# Autodesk Inventor assembly: Custom Cover Full Assembly_2
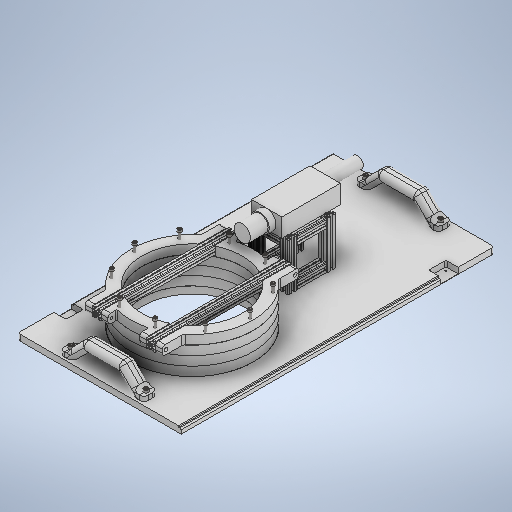
[picture p0: Inventor's stored thumbnail of the model, 512x512]
Saved by Autodesk Inventor 2025 (Build 290162000, 162)
## iProperties
Created: 2024-04-26
Part Number: Custom Cover Full Assembly_2
Document SubType Name: Assembly
Designer: Thienan Hoang
Author: Thienan Hoang
## Documents named in this file (13)
- C:\GitHub\In-situ-monitoring-of-powder-bed-fusion-additive-manufacturing\system_development\Orichalcum\v0.2\Hardware_design\custom-cover\Custom Cover Full Assembly_2-fs.iam
- C:\GitHub\In-situ-monitoring-of-powder-bed-fusion-additive-manufacturing\system_development\Orichalcum\v0.2\Hardware_design\custom-cover\cover\Updated Cover.ipt
- C:\Users\mayhe\OneDrive\Documents\GitHub\In-situ-monitoring-of-powder-bed-fusion-additive-manufacturing\system_development\Orichalcum\v0.1\Hardware_design\galvo-scanner\GVS102.iam
- C:\GitHub\In-situ-monitoring-of-powder-bed-fusion-additive-manufacturing\system_development\Orichalcum\v0.2\Hardware_design\custom-cover\cylinder-parts\cylinder-segments\Head Thing.ipt
- C:\Users\mayhe\OneDrive\Documents\GitHub\In-situ-monitoring-of-powder-bed-fusion-additive-manufacturing\system_development\Orichalcum\v0.1\Hardware_design\custom-cover\cylinder-parts\final-parts\Cylinder Bottom.ipt
- C:\GitHub\In-situ-monitoring-of-powder-bed-fusion-additive-manufacturing\system_development\Orichalcum\v0.2\Hardware_design\custom-cover\cover\Handles.ipt
- C:\GitHub\In-situ-monitoring-of-powder-bed-fusion-additive-manufacturing\system_development\Orichalcum\v0.2\Hardware_design\custom-cover\8020-parts\ANSI B18.3.1M - M6x1 x 20(1).ipt
- C:\GitHub\In-situ-monitoring-of-powder-bed-fusion-additive-manufacturing\system_development\Orichalcum\v0.2\Hardware_design\custom-cover\8020-parts\ANSI B18.3.1M - M5x0.8 x 100(1).ipt
- C:\GitHub\In-situ-monitoring-of-powder-bed-fusion-additive-manufacturing\system_development\Orichalcum\v0.2\Hardware_design\custom-cover\cylinder-parts\Cylinder Spacer (x3).ipt
- C:\GitHub\In-situ-monitoring-of-powder-bed-fusion-additive-manufacturing\system_development\Orichalcum\v0.2\Hardware_design\custom-cover\cylinder-parts\Cylinder 80-20 Spacer_1.ipt
- C:\GitHub\In-situ-monitoring-of-powder-bed-fusion-additive-manufacturing\system_development\Orichalcum\v0.2\Hardware_design\custom-cover\cylinder-parts\Cylinder 80-20 Spacer_2.ipt
- C:\GitHub\In-situ-monitoring-of-powder-bed-fusion-additive-manufacturing\system_development\Orichalcum\v0.2\Hardware_design\custom-cover\8020-parts\20-2020-300.ipt
- C:\GitHub\In-situ-monitoring-of-powder-bed-fusion-additive-manufacturing\system_development\Orichalcum\v0.2\Hardware_design\custom-cover\LaserFrameAssembly.iam
## Components (30 placed, 12 different names)
1. Updated Cover:1 — Flush:5, Mate:48, Mate:98, Mate:106, Mate:107, Mate:108, Mate:109, Mate:128, Mate:129
2. GVS102:1 [sub-assembly]
3. Head Thing:1
4. Cylinder Bottom:1 — Mate:98
5. Handles:1 — Mate:108, Mate:109, Insert:18, Insert:19
6. Handles:2 — Mate:106, Mate:107, Insert:20, Insert:21
7. Cylinder Spacer (x3):1 — Rotational:1, Mate:128
8. Cylinder Spacer (x3):2 — Rotational:1, Rotational:2
9. Cylinder Spacer (x3):3 — Rotational:2, Mate:127
10. Cylinder 80-20 Spacer_1:1 — Flush:9, Flush:10, Mate:123, Mate:126, Flush:15, Flush:16
11. Cylinder 80-20 Spacer_2:1 — Mate:122, Flush:7, Flush:8
12. 20-2020-300:1 — Mate:122, Flush:7, Flush:8, Flush:9, Flush:10, Mate:123
13. Cylinder 80-20 Spacer_1:2
14. Cylinder 80-20 Spacer_2:2 — Mate:127
15. 20-2020-300:2 — Mate:126, Flush:15, Flush:16
16. LaserFrameAssembly:1 [sub-assembly] — Mate:129
17. Forged Socket Head Cap Screw - Metric M6x1 x 20:1 — Insert:18
18. Forged Socket Head Cap Screw - Metric M6x1 x 20:2 — Insert:19
19. Forged Socket Head Cap Screw - Metric M6x1 x 20:3 — Insert:20
20. Forged Socket Head Cap Screw - Metric M6x1 x 20:4 — Insert:21
21. Forged Socket Head Cap Screw - Metric M5x0.8 x 100:1
22. Forged Socket Head Cap Screw - Metric M5x0.8 x 100:3
23. Forged Socket Head Cap Screw - Metric M5x0.8 x 100:4
24. Forged Socket Head Cap Screw - Metric M5x0.8 x 100:5
25. Forged Socket Head Cap Screw - Metric M5x0.8 x 100:6
26. Forged Socket Head Cap Screw - Metric M5x0.8 x 100:7
27. Forged Socket Head Cap Screw - Metric M5x0.8 x 100:8
28. Forged Socket Head Cap Screw - Metric M5x0.8 x 100:9
29. Forged Socket Head Cap Screw - Metric M5x0.8 x 100:10
30. Forged Socket Head Cap Screw - Metric M5x0.8 x 100:11
## Relationships (32: Mate 14, Flush 12, Insert 4, RevoluteJoint 2)
- Flush:5 (180 mm): Updated Cover:1
- Mate:48: Updated Cover:1
- Flush:6 (38 mm)
- Mate:98: Updated Cover:1 ↔ Cylinder Bottom:1
- Mate:106: Updated Cover:1 ↔ Handles:2
- Mate:107: Updated Cover:1 ↔ Handles:2
- Mate:108: Updated Cover:1 ↔ Handles:1
- Mate:109: Updated Cover:1 ↔ Handles:1
- Insert:18: Handles:1 ↔ Forged Socket Head Cap Screw - Metric M6x1 x 20:1
- Insert:19: Handles:1 ↔ Forged Socket Head Cap Screw - Metric M6x1 x 20:2
- Insert:20: Handles:2 ↔ Forged Socket Head Cap Screw - Metric M6x1 x 20:3
- Insert:21: Handles:2 ↔ Forged Socket Head Cap Screw - Metric M6x1 x 20:4
- Rotational:1 [RevoluteJoint]: Cylinder Spacer (x3):1 ↔ Cylinder Spacer (x3):2
- Rotational:2 [RevoluteJoint]: Cylinder Spacer (x3):2 ↔ Cylinder Spacer (x3):3
- Mate:122: Cylinder 80-20 Spacer_2:1 ↔ 20-2020-300:1
- Flush:7: Cylinder 80-20 Spacer_2:1 ↔ 20-2020-300:1
- Flush:8: Cylinder 80-20 Spacer_2:1 ↔ 20-2020-300:1
- Flush:9: Cylinder 80-20 Spacer_1:1 ↔ 20-2020-300:1
- Flush:10: Cylinder 80-20 Spacer_1:1 ↔ 20-2020-300:1
- Mate:123: Cylinder 80-20 Spacer_1:1 ↔ 20-2020-300:1
- [Mate]: Cylinder 80-20 Spacer_2:2 ↔ 20-2020-300:2
- [Flush]: Cylinder 80-20 Spacer_2:2 ↔ 20-2020-300:2
- [Flush]: Cylinder 80-20 Spacer_2:2 ↔ 20-2020-300:2
- [Flush]: Cylinder 80-20 Spacer_1:2 ↔ 20-2020-300:2
- [Flush]: Cylinder 80-20 Spacer_1:2 ↔ 20-2020-300:2
- [Mate]: Cylinder 80-20 Spacer_1:2 ↔ 20-2020-300:2
- Mate:126: Cylinder 80-20 Spacer_1:1 ↔ 20-2020-300:2
- Flush:15: Cylinder 80-20 Spacer_1:1 ↔ 20-2020-300:2
- Flush:16: Cylinder 80-20 Spacer_1:1 ↔ 20-2020-300:2
- Mate:127: Cylinder Spacer (x3):3 ↔ Cylinder 80-20 Spacer_2:2
- Mate:128: Updated Cover:1 ↔ Cylinder Spacer (x3):1
- Mate:129: Updated Cover:1 ↔ LaserFrameAssembly:1
## Named parameters: d405_d399 = 0 mm, d406_d400 = 0 mm, d407_d401 = 0 mm, d408_d402 = 0 mm, d409_d403 = 0 mm, d410_d404 = 0 mm
